# Autodesk Inventor assembly: STI Hybrid 98 Cryocooler Assembly
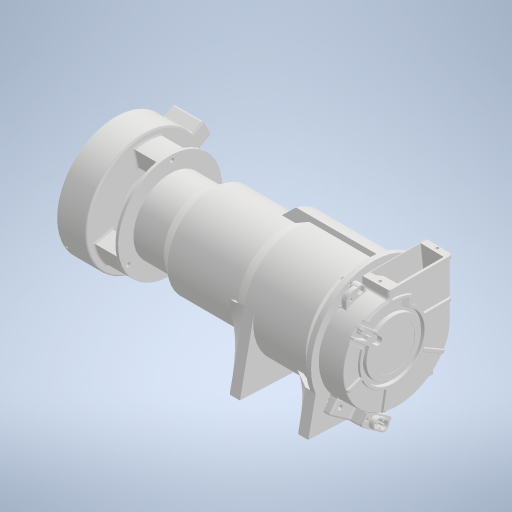
[picture p0: Inventor's stored thumbnail of the model, 512x512]
Saved by Autodesk Inventor 2023 (Build 270158000, 158)
## iProperties
Created: 2024-05-02
Part Number: STI Hybrid 98 Cryocooler Assembly
Document SubType Name: Assembly
Designer: incep
Author: incep
## Documents named in this file (7)
- C:\Users\incep\OneDrive\Desktop\3D Printer Stuff\CryocoolerHybrid98\STI Hybrid 98 Cryocooler Assembly.iam
- C:\Users\incep\OneDrive\Desktop\3D Printer Stuff\CryocoolerHybrid98\STI Hybrid 98 Cryocooler.ipt
- C:\Users\incep\OneDrive\Desktop\3D Printer Stuff\CryocoolerHybrid98\STI Hybrid 98 Cooling Shroud.ipt
- C:\Users\incep\OneDrive\Desktop\3D Printer Stuff\CryocoolerHybrid98\OAB800AN_m0.ipt
- C:\Users\incep\OneDrive\Desktop\3D Printer Stuff\CryocoolerHybrid98\BlowerPowerEntry.ipt
- C:\Users\incep\OneDrive\Desktop\3D Printer Stuff\CryocoolerHybrid98\e_0100.3017a003.ipt
- C:\Users\incep\OneDrive\Desktop\3D Printer Stuff\CryocoolerHybrid98\Dewar-YDS-3-Adapter.ipt
## Components (6 placed, 6 different names)
1. STI Hybrid 98 Cryocooler:1 — Flush:1, Flush:2, Flush:3, Mate:1, Mate:2, Mate:3, Mate:4, Mate:5, Flush:4, Flush:5, Mate:6, Mate:7, Mate:15, Mate:18
2. STI Hybrid 98 Cooling Shroud:1 — Mate:5, Flush:4, Flush:5, Mate:6, Mate:7, Mate:8, Mate:9, Mate:17
3. OAB800AN_m0:1 — Mate:8, Mate:9, Angle:1, Mate:13, Mate:14, Angle:2
4. BlowerPowerEntry:1 — Mate:10, Mate:11, Mate:12, Mate:13, Mate:14, Angle:2
5. e_0100.3017a003:1 — Mate:10, Mate:11, Mate:12
6. Dewar-YDS-3-Adapter:1 — Mate:15, Mate:17, Mate:18
## Relationships (24: Mate 17, Flush 5, Angle 2)
- Flush:1: STI Hybrid 98 Cryocooler:1
- Flush:2: STI Hybrid 98 Cryocooler:1
- Flush:3: STI Hybrid 98 Cryocooler:1
- Mate:1: STI Hybrid 98 Cryocooler:1
- Mate:2: STI Hybrid 98 Cryocooler:1
- Mate:3: STI Hybrid 98 Cryocooler:1
- Mate:4: STI Hybrid 98 Cryocooler:1
- Mate:5: STI Hybrid 98 Cryocooler:1 ↔ STI Hybrid 98 Cooling Shroud:1
- Flush:4: STI Hybrid 98 Cryocooler:1 ↔ STI Hybrid 98 Cooling Shroud:1
- Flush:5: STI Hybrid 98 Cryocooler:1 ↔ STI Hybrid 98 Cooling Shroud:1
- Mate:6: STI Hybrid 98 Cryocooler:1 ↔ STI Hybrid 98 Cooling Shroud:1
- Mate:7: STI Hybrid 98 Cryocooler:1 ↔ STI Hybrid 98 Cooling Shroud:1
- Mate:8: STI Hybrid 98 Cooling Shroud:1 ↔ OAB800AN_m0:1
- Mate:9: STI Hybrid 98 Cooling Shroud:1 ↔ OAB800AN_m0:1
- Angle:1 (0 deg): OAB800AN_m0:1
- Mate:10: BlowerPowerEntry:1 ↔ e_0100.3017a003:1
- Mate:11: BlowerPowerEntry:1 ↔ e_0100.3017a003:1
- Mate:12: BlowerPowerEntry:1 ↔ e_0100.3017a003:1
- Mate:13: OAB800AN_m0:1 ↔ BlowerPowerEntry:1
- Mate:14: OAB800AN_m0:1 ↔ BlowerPowerEntry:1
- Angle:2 (325 deg): OAB800AN_m0:1 ↔ BlowerPowerEntry:1
- Mate:15: STI Hybrid 98 Cryocooler:1 ↔ Dewar-YDS-3-Adapter:1
- Mate:17: STI Hybrid 98 Cooling Shroud:1 ↔ Dewar-YDS-3-Adapter:1
- Mate:18: STI Hybrid 98 Cryocooler:1 ↔ Dewar-YDS-3-Adapter:1
